# Autodesk Inventor assembly: estructura hombro brazo
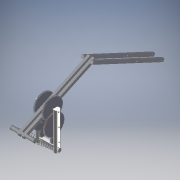
[picture p0: Inventor's stored thumbnail of the model, 180x180]
Saved by Autodesk Inventor 2016 (Build 200138000, 138)
## iProperties
Created: 2016-05-28
Part Number: estructura hombro brazo
Document SubType Name: Assembly
Designer: Admin
Author: Admin
## Documents named in this file (16)
- C:\Users\Admin\Desktop\dimer hackaday inventor\estructura hombro brazo.iam
- C:\Users\Admin\Desktop\dimer hackaday inventor\Part1.ipt
- C:\Users\Admin\Desktop\dimer hackaday inventor\Part3.ipt
- C:\Users\Admin\Desktop\dimer hackaday inventor\eje hombro.iam
- C:\Users\Admin\Desktop\dimer hackaday inventor\eje pequeño.iam
- C:\Users\Admin\Desktop\dimer hackaday inventor\engranajes hombro.iam
- C:\Users\Admin\Desktop\dimer hackaday inventor\engranaje pequeño.iam
- C:\Users\Admin\Desktop\dimer hackaday inventor\engranajes hombro_CPY.iam
- C:\Users\Admin\Desktop\dimer hackaday inventor\engranaje pequeño_CPY.iam
- C:\Users\Admin\Desktop\dimer hackaday inventor\engranajes hombro_CPY_MIR.iam
- C:\Users\Admin\Desktop\dimer hackaday inventor\engranaje pequeño_CPY_MIR.iam
- C:\Users\Admin\Desktop\dimer hackaday inventor\barra horizontal hombro.iam
- C:\Users\Admin\Desktop\dimer hackaday inventor\barra horizontal hombro_MIR.iam
- C:\Users\Admin\Desktop\dimer hackaday inventor\muelles hombro2.ipt
- C:\Users\Admin\Desktop\dimer hackaday inventor\muelles hombro2_MIR.ipt
- C:\Users\Admin\Desktop\dimer hackaday inventor\barra horizontal hombro_MIR1.iam
## Components (22 placed, 15 different names)
1. Part3:1 — Flush:3, Mate:1, Flush:4
2. eje hombro:1 [sub-assembly] — Mate:18, Mate:19, Mate:20, Mate:23
3. eje pequeño:1 [sub-assembly] — Flush:5, Mate:10, Mate:14, Mate:16
4. eje pequeño:2 [sub-assembly] — Mate:12, Flush:6
5. engranajes hombro_CPY:1 [sub-assembly] — Flush:8, Tangent:2, Mate:18, Rotation:6, Mate:21, Rotation:8
6. engranaje pequeño_CPY:1 [sub-assembly] — Flush:8, Tangent:2, Mate:14, Mate:15, Rotation:4, Rotation:6
7. engranajes hombro_CPY_MIR:1 [sub-assembly] — Tangent:3, Flush:9, Rotation:7, Mate:19, Mate:22
8. engranaje pequeño_CPY_MIR:1 [sub-assembly] — Tangent:3, Flush:9, Mate:16, Mate:17, Rotation:5, Rotation:7
9. barra horizontal hombro:1 [sub-assembly] — Mate:20, Mate:21, Rotation:8, Mate:34, Mate:38
10. barra horizontal hombro_MIR:1 [sub-assembly] — Mate:22, Mate:23, Mate:33, Mate:35, Mate:39
11. muelles hombro2:1 — Mate:32, Mate:35
12. eje pequeño:3 [sub-assembly] — Mate:37
13. eje pequeño:4 [sub-assembly] — Mate:32, Mate:36, Mate:37
14. muelles hombro2_MIR:1 — Mate:33, Mate:34, Mate:36
15. barra horizontal hombro:3 [sub-assembly] — Mate:38, Flush:10, Flush:11
16. barra horizontal hombro_MIR1:1 [sub-assembly] — Mate:39, Flush:10, Flush:11
17. Part1:1 — Flush:3, Mate:1, Flush:4, Flush:5, Flush:6
18. Part1:2 — Mate:13
19. engranajes hombro:1 [sub-assembly] — Mate:10, Tangent:1, Rotation:1, Flush:7, Mate:15, Rotation:4
20. engranaje pequeño:1 [sub-assembly] — Tangent:1, Mate:12, Rotation:1, Flush:7, Mate:13
21. engranajes hombro:2 [sub-assembly] — Mate:17, Rotation:5
22. engranaje pequeño:2 [sub-assembly]
## Component patterns: (2 elements, first: Part1:1), (2 elements, first: engranajes hombro:1 + engranaje pequeño:1)
## Relationships (40: Mate 22, Flush 9, RelateRotation 6, Tangent 3)
- Flush:3: Part3:1 ↔ Part1:1
- Mate:1 (-2 mm): Part3:1 ↔ Part1:1
- Flush:4: Part3:1 ↔ Part1:1
- Flush:5 (-5 mm): eje pequeño:1 ↔ Part1:1
- Mate:10: eje pequeño:1 ↔ engranajes hombro:1
- Mate:12: eje pequeño:2 ↔ engranaje pequeño:1
- Tangent:1: engranajes hombro:1 ↔ engranaje pequeño:1
- Flush:6 (-5 mm): eje pequeño:2 ↔ Part1:1
- Rotation:1 [RelateRotation] (3 ul): engranajes hombro:1 ↔ engranaje pequeño:1
- Flush:7: engranajes hombro:1 ↔ engranaje pequeño:1
- Mate:13 (5 mm): Part1:2 ↔ engranaje pequeño:1
- Flush:8 (1 mm): engranajes hombro_CPY:1 ↔ engranaje pequeño_CPY:1
- Tangent:2: engranajes hombro_CPY:1 ↔ engranaje pequeño_CPY:1
- Mate:14: eje pequeño:1 ↔ engranaje pequeño_CPY:1
- Mate:15: engranaje pequeño_CPY:1 ↔ engranajes hombro:1
- Tangent:3: engranajes hombro_CPY_MIR:1 ↔ engranaje pequeño_CPY_MIR:1
- Flush:9 (1 mm): engranajes hombro_CPY_MIR:1 ↔ engranaje pequeño_CPY_MIR:1
- Mate:16: eje pequeño:1 ↔ engranaje pequeño_CPY_MIR:1
- Mate:17: engranaje pequeño_CPY_MIR:1 ↔ engranajes hombro:2
- Rotation:4 [RelateRotation] (1 ul): engranaje pequeño_CPY:1 ↔ engranajes hombro:1
- Rotation:5 [RelateRotation] (1 ul): engranaje pequeño_CPY_MIR:1 ↔ engranajes hombro:2
- Mate:18: eje hombro:1 ↔ engranajes hombro_CPY:1
- Rotation:6 [RelateRotation] (3 ul): engranajes hombro_CPY:1 ↔ engranaje pequeño_CPY:1
- Rotation:7 [RelateRotation] (3 ul): engranajes hombro_CPY_MIR:1 ↔ engranaje pequeño_CPY_MIR:1
- Mate:19: eje hombro:1 ↔ engranajes hombro_CPY_MIR:1
- Mate:20: eje hombro:1 ↔ barra horizontal hombro:1
- Mate:21: engranajes hombro_CPY:1 ↔ barra horizontal hombro:1
- Rotation:8 [RelateRotation] (1 ul): engranajes hombro_CPY:1 ↔ barra horizontal hombro:1
- Mate:22: engranajes hombro_CPY_MIR:1 ↔ barra horizontal hombro_MIR:1
- Mate:23: eje hombro:1 ↔ barra horizontal hombro_MIR:1
- Mate:32: muelles hombro2:1 ↔ eje pequeño:4
- Mate:33: barra horizontal hombro_MIR:1 ↔ muelles hombro2_MIR:1
- Mate:34: barra horizontal hombro:1 ↔ muelles hombro2_MIR:1
- Mate:35: barra horizontal hombro_MIR:1 ↔ muelles hombro2:1
- Mate:36: eje pequeño:4 ↔ muelles hombro2_MIR:1
- Mate:37: eje pequeño:3 ↔ eje pequeño:4
- Mate:38: barra horizontal hombro:1 ↔ barra horizontal hombro:3
- Mate:39: barra horizontal hombro_MIR:1 ↔ barra horizontal hombro_MIR1:1
- Flush:10: barra horizontal hombro:3 ↔ barra horizontal hombro_MIR1:1
- Flush:11: barra horizontal hombro:3 ↔ barra horizontal hombro_MIR1:1
